# Autodesk Inventor assembly: Assembly146-01
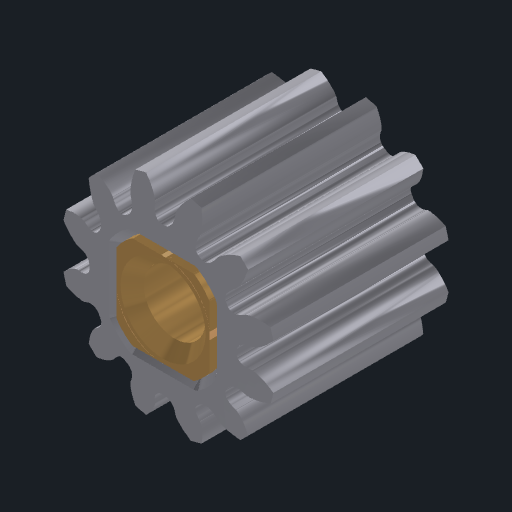
[picture p0: Inventor's stored thumbnail of the model, 512x512]
Saved by Autodesk Inventor 2023.2 (Build 272271000, 271)
## iProperties
Created: 2022-08-02
Part Number: Assembly146-01
Document SubType Name: Assembly
Designer: ylu12
Author: ylu12
## Documents named in this file (31)
- D:\CAD\Parts\standard\Motion\Gears\HS\HS Gear.iam
- D:\CAD\Parts\standard\Motion\Adapters\HS Shaft Adapter Circle.ipt
- D:\CAD\Parts\standard\Motion\Adapters\HS Shaft Adapter Square.ipt
- D:\CAD\Parts\standard\Motion\Gears\HS\Reference parts\HS 12T Gear, No Insert.ipt
- D:\CAD\Parts\standard\Motion\Gears\HS\Reference parts\HS 24T Gear, No Insert.ipt
- D:\CAD\Parts\standard\Motion\Gears\HS\Reference parts\HS 36T Gear, No Insert.ipt
- D:\CAD\Parts\standard\Motion\Gears\HS\Reference parts\HS 48T Gear, No Insert.ipt
- D:\CAD\Parts\standard\Motion\Gears\HS\Reference parts\HS 60T Gear, No Insert.ipt
- D:\CAD\Parts\standard\Motion\Gears\HS\Reference parts\HS 72T Gear, No Insert.ipt
- D:\CAD\Parts\standard\Motion\Gears\HS\Reference parts\HS 84T Gear, No Insert.ipt
- HS 12T Gear, Circle.iam
- HS 12T Gear, No Insert.iam
- HS 12T Gear, Square.iam
- HS 24T Gear, Circle.iam
- HS 24T Gear, No Insert.iam
- HS 24T Gear, Square.iam
- HS 36T Gear, Circle.iam
- HS 36T Gear, No Insert.iam
- HS 36T Gear, Square.iam
- HS 48T Gear, Circle.iam
- HS 48T Gear, No Insert.iam
- HS 48T Gear, Square.iam
- HS 60T Gear, Circle.iam
- HS 60T Gear, No Insert.iam
- HS 60T Gear, Square.iam
- HS 72T Gear, Circle.iam
- HS 72T Gear, No Insert.iam
- HS 72T Gear, Square.iam
- HS 84T Gear, Circle.iam
- HS 84T Gear, No Insert.iam
- HS 84T Gear, Square.iam
## Components (9 placed, 9 different names)
1. Circle — Mate:1, Mate:2, Flush:1
2. Square — Mate:3, Mate:4, Flush:2
3. 12T — Mate:5, Mate:6, Flush:3
4. 24T — Mate:7, Mate:8, Flush:4
5. 36T — Flush:5, Mate:9, Mate:10
6. 48T — Flush:6, Mate:11, Mate:12
7. 60T — Flush:7, Mate:13, Mate:14
8. 72T — Flush:8, Mate:15, Mate:16
9. 84T — Flush:9, Mate:17, Mate:18
## Relationships (27: Mate 18, Flush 9)
- Mate:1: Circle
- Mate:2: Circle
- Flush:1 (6.35 mm): Circle
- Mate:3: Square
- Mate:4: Square
- Flush:2 (6.35 mm): Square
- Mate:5: 12T
- Mate:6: 12T
- Flush:3: 12T
- Mate:7: 24T
- Mate:8: 24T
- Flush:4: 24T
- Flush:5: 36T
- Flush:6: 48T
- Flush:7: 60T
- Flush:8: 72T
- Flush:9: 84T
- Mate:9: 36T
- Mate:10: 36T
- Mate:11: 48T
- Mate:12: 48T
- Mate:13: 60T
- Mate:14: 60T
- Mate:15: 72T
- Mate:16: 72T
- Mate:17: 84T
- Mate:18: 84T
